# Autodesk Inventor assembly: linia
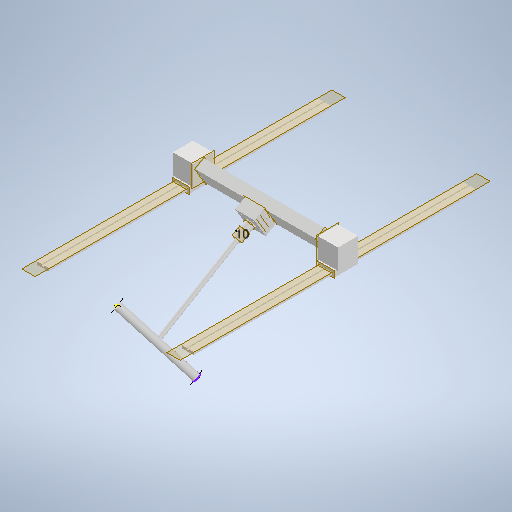
[picture p0: Inventor's stored thumbnail of the model, 512x512]
Saved by Autodesk Inventor 2025.1 (Build 291241000, 241)
## iProperties
Created: 2024-11-25
Part Number: linia
Document SubType Name: Assembly
Designer: dell
Author: dell
## Documents named in this file (5)
- D:\creap\prot_tonbo\prot_Tonbo.iam
- D:\creap\prot_tonbo\block1.ipt
- D:\creap\prot_tonbo\moto1.ipt
- D:\creap\Tonbo.iam
- D:\creap\prot_tonbo\linear_guide.iam
## Components (6 placed, 4 different names)
1. moto1:2 — 回転:1, リジッド:2
2. moto1:3 — 回転:2, リジッド:3
3. block1:1 — 回転:1, 回転:2, リジッド:4
4. Tonbo:1 [sub-assembly] — リジッド:4
5. linear_guide:1 [sub-assembly] — リジッド:3
6. linear_guide:2 [sub-assembly] — リジッド:2
## Relationships (5: WeldJoint 3, RevoluteJoint 2)
- 回転:1 [RevoluteJoint]: moto1:2 ↔ block1:1
- 回転:2 [RevoluteJoint]: moto1:3 ↔ block1:1
- リジッド:2 [WeldJoint]: moto1:2 ↔ linear_guide:2
- リジッド:3 [WeldJoint] (-50 mm): moto1:3 ↔ linear_guide:1
- リジッド:4 [WeldJoint]: block1:1 ↔ Tonbo:1
